# Autodesk Inventor assembly: 2016-01-27-RhinoRobotV03
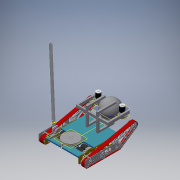
[picture p0: Inventor's stored thumbnail of the model, 180x180]
Saved by Autodesk Inventor 2016 SP1 (Build 200210100, 210)
## iProperties
Created: 2016-01-23
Part Number: 2016-01-27-RhinoRobotV03
Document SubType Name: Assembly
Designer: steele
Mass: 10784.8 g
Surface Area: 26494.6 cm^2
Volume: 9600.19 cm^3
Density: 1.12339 g/cm^3
Author: steele
## Documents named in this file (9)
- C:\snobotics\CAD-Development\robSteele\SnoBotics2016\2016-01-28-RhinoRobot\2016-01-27-RhinoRobotV03.iam
- C:\snobotics\CAD-Development\robSteele\SnoBotics2016\RhinoTrackDriveModule\am-3322+RhinoTrackDriveModule.iam
- C:\snobotics\CAD-Development\robSteele\SnoBotics2016\TelescopeArm\TelescopingArm.iam
- C:\snobotics\CAD-Development\robSteele\SnoBotics2016\2016-01-26-RhinoRobot\maxAllowedVolume.ipt
- C:\snobotics\CAD-Development\robSteele\SnoBotics2016\AM Parts\SnowBlowerMotorAndHub.iam
- C:\snobotics\CAD-Development\robSteele\SnoBotics2016\TelescopeArm\WoodPully.ipt
- C:\snobotics\CAD-Development\robSteele\SnoBotics2016\2016-01-28-BallShooter\BallShooterV03.iam
- C:\snobotics\CAD-Development\robSteele\SnoBotics2016\RhinoBottomFloorOptions\RhinoBottomFloorPlate04.ipt
- C:\snobotics\CAD-Development\robSteele\SnoBotics2016\RhinoTrackDriveModule\am-3322+RhinoTrackDriveModule_MIR8.iam
## Components (8 placed, 8 different names)
1. RhinoBottomFloorPlate04:1 — Mate:1, Flush:2, Flush:3, Flush:5, Flush:7, Mate:11, Mate:14, Mate:15, Flush:9, Mate:16, Flush:11, Mate:17
2. am-3322+RhinoTrackDriveModule:1 [sub-assembly] — Mate:1, Flush:2, Flush:3, Mate:6, Mate:10
3. maxAllowedVolume:1 — Mate:4, Mate:6, Flush:5
4. TelescopingArm:1 [sub-assembly] — Mate:10, Flush:7, Mate:11
5. SnowBlowerMotorAndHub:1 [sub-assembly] — Mate:14, Mate:15, Flush:9, Insert:1
6. WoodPully:1 — Insert:1
7. BallShooterV03:1 [sub-assembly] — Mate:16, Flush:11, Mate:17
8. am-3322+RhinoTrackDriveModule_MIR8:1 [sub-assembly]
## Relationships (16: Mate 9, Flush 6, Insert 1)
- Mate:1 (3.175 mm): RhinoBottomFloorPlate04:1 ↔ am-3322+RhinoTrackDriveModule:1
- Flush:2: RhinoBottomFloorPlate04:1 ↔ am-3322+RhinoTrackDriveModule:1
- Flush:3: RhinoBottomFloorPlate04:1 ↔ am-3322+RhinoTrackDriveModule:1
- Mate:4: maxAllowedVolume:1
- Mate:6: am-3322+RhinoTrackDriveModule:1 ↔ maxAllowedVolume:1
- Flush:5 (-381 mm): RhinoBottomFloorPlate04:1 ↔ maxAllowedVolume:1
- Mate:10: am-3322+RhinoTrackDriveModule:1 ↔ TelescopingArm:1
- Flush:7: RhinoBottomFloorPlate04:1 ↔ TelescopingArm:1
- Mate:11 (25.4 mm): RhinoBottomFloorPlate04:1 ↔ TelescopingArm:1
- Mate:14: RhinoBottomFloorPlate04:1 ↔ SnowBlowerMotorAndHub:1
- Mate:15: RhinoBottomFloorPlate04:1 ↔ SnowBlowerMotorAndHub:1
- Flush:9: RhinoBottomFloorPlate04:1 ↔ SnowBlowerMotorAndHub:1
- Insert:1: SnowBlowerMotorAndHub:1 ↔ WoodPully:1
- Mate:16 (-152.4 mm): RhinoBottomFloorPlate04:1 ↔ BallShooterV03:1
- Flush:11: RhinoBottomFloorPlate04:1 ↔ BallShooterV03:1
- Mate:17: RhinoBottomFloorPlate04:1 ↔ BallShooterV03:1
## Named parameters: robotWidth = 660.4 mm, halfRobotWidth = 330.2 mm, maxPerimeter = 3048 mm, maxLength = 863.6 mm, widthOfTrack = 95.25 mm, boardWidth = 469.9 mm
